# Autodesk Inventor assembly: Колесо 2 в сборе
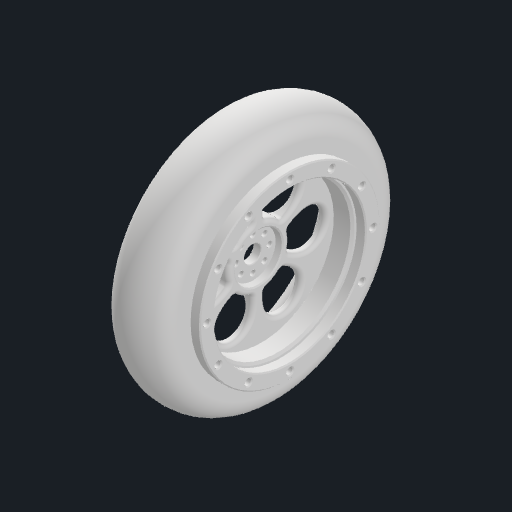
[picture p0: Inventor's stored thumbnail of the model, 512x512]
Saved by Autodesk Inventor 2025 (Build 290162010, 162A)
## iProperties
Created: 2025-01-14
Part Number: Колесо 2 в сборе
Document SubType Name: Assembly
Designer: Edward_Higgins
Author: Edward_Higgins
## Documents named in this file (4)
- D:\Users\Edward_Higgins\Desktop\ZAVOD\Робот Сколково\Колесо 2 в сборе.iam
- D:\Users\Edward_Higgins\Desktop\ZAVOD\Робот Сколково\Колесо 2 .ipt
- D:\Users\Edward_Higgins\Desktop\ZAVOD\Робот Сколково\Ступица.ipt
- D:\Users\Edward_Higgins\Desktop\ZAVOD\Робот Сколково\Фланец колеса.ipt
## Components (3 placed, 3 different names)
1. Колесо 2 :1 — Совмещение:1, Совмещение:2, Совмещение:3, Совмещение:4, Совмещение:7, Совмещение:8, Совмещение:9, Совмещение:10
2. Ступица:1 — Совмещение:3, Совмещение:4, Совмещение:8
3. Фланец колеса:1 — Совмещение:7, Совмещение:9, Совмещение:10
## Relationships (8: Mate 8)
- Совмещение:1 [Mate]: Колесо 2 :1
- Совмещение:2 [Mate]: Колесо 2 :1
- Совмещение:3 [Mate]: Колесо 2 :1 ↔ Ступица:1
- Совмещение:4 [Mate]: Колесо 2 :1 ↔ Ступица:1
- Совмещение:7 [Mate]: Колесо 2 :1 ↔ Фланец колеса:1
- Совмещение:8 [Mate]: Колесо 2 :1 ↔ Ступица:1
- Совмещение:9 [Mate]: Колесо 2 :1 ↔ Фланец колеса:1
- Совмещение:10 [Mate]: Колесо 2 :1 ↔ Фланец колеса:1
